# Autodesk Inventor assembly: Assembly1
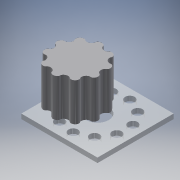
[picture p0: Inventor's stored thumbnail of the model, 180x180]
Saved by Autodesk Inventor 2019 (Build 230136000, 136)
## iProperties
Created: 2019-05-17
Part Number: Assembly1
Document SubType Name: Assembly
Designer: Alex Jones
Author: Alex Jones
## Documents named in this file (3)
- C:\Users\Alex Jones\Documents\Inventor\cylcoid\Assembly1.iam
- C:\Users\Alex Jones\Documents\Inventor\cylcoid\basePlate.ipt
- C:\Users\Alex Jones\Documents\Inventor\CNC\gear.ipt
## Components (2 placed, 2 different names)
1. basePlate:1 — Mate:1
2. gear:1 — Mate:1
## Relationships (1: Mate 1)
- Mate:1: basePlate:1 ↔ gear:1
